# Autodesk Inventor assembly: ASY TZS FDS way1_940
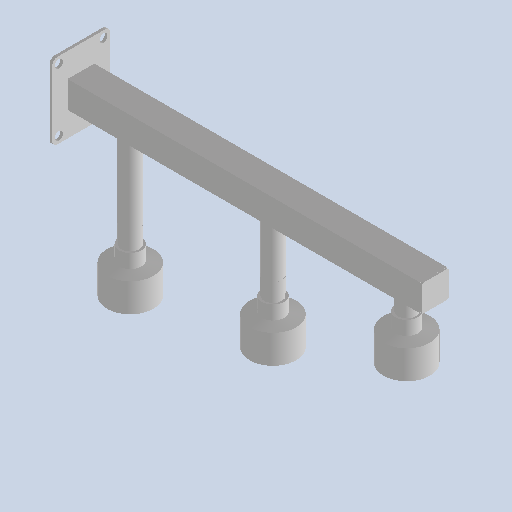
[picture p0: Inventor's stored thumbnail of the model, 512x512]
Saved by Autodesk Inventor 2025 (Build 290162010, 162A)
## iProperties
Created: 2025-07-02
Part Number: ASY TZS FDS way1_940
Document SubType Name: Assembly
Designer: admin
Author: user
## Documents named in this file (8)
- C:\Users\pokla\Documents\Inventor\TZS-Tazovskiy\Filter D940\FDS 940\ASY TZS FDS way1_940.iam
- C:\Users\pokla\Documents\Inventor\TZS-Tazovskiy\Filter D940\FDS 940\TZS 1661 FDS 940 way tube 1.ipt
- C:\Users\pokla\Documents\Inventor\TZS-Tazovskiy\Filter D940\FDS 940\TZS dummy filter element_940.ipt
- C:\Users\pokla\Documents\Inventor\TZS-Tazovskiy\Filter D940\FDS 940\TZS dummy pipe nippel_940.ipt
- C:\Users\pokla\Documents\Inventor\TZS-Tazovskiy\Filter D940\FDS 940\TZS 1684 FDS 940 way tube 4.ipt
- C:\Users\pokla\Documents\Inventor\TZS-Tazovskiy\Filter D940\FDS 940\TZS 1686 FDS 940 way tube 6.ipt
- C:\Users\pokla\Documents\Inventor\TZS-Tazovskiy\Filter D940\FDS 940\TZS 1669 FDS 940 FLANGE 3.ipt
- C:\Users\pokla\Documents\Inventor\TZS-Tazovskiy\Filter D940\FDS 940\TZS 1666 FDS 940 CUP 1.ipt
## Components (11 placed, 7 different names)
1. TZS 1661 FDS 940 way tube 1.ipt:1 — Rigid:2, Rigid:5, Rigid:10, Rigid:12, Rigid:13
2. TZS dummy filter element_940.ipt:1 — Rigid:1
3. TZS dummy pipe nippel_940.ipt:1 — Rigid:2, Rigid:1
4. TZS 1684 FDS 940 way tube 4.ipt:1 — Rigid:5, Rigid:4
5. TZS dummy filter element_940.ipt:2 — Rigid:3
6. TZS dummy pipe nippel_940.ipt:2 — Rigid:4, Rigid:3
7. TZS 1686 FDS 940 way tube 6.ipt:1 — Rigid:10, Rigid:7
8. TZS dummy filter element_940.ipt:3 — Rigid:6
9. TZS dummy pipe nippel_940.ipt:3 — Rigid:7, Rigid:6
10. TZS 1669 FDS 940 FLANGE 3.ipt:1 — Rigid:12
11. TZS 1666 FDS 940 CUP 1.ipt:1 — Rigid:13
## Relationships (10: WeldJoint 10)
- Rigid:2 [WeldJoint]: TZS 1661 FDS 940 way tube 1.ipt:1 ↔ TZS dummy pipe nippel_940.ipt:1
- Rigid:1 [WeldJoint]: TZS dummy filter element_940.ipt:1 ↔ TZS dummy pipe nippel_940.ipt:1
- Rigid:5 [WeldJoint]: TZS 1661 FDS 940 way tube 1.ipt:1 ↔ TZS 1684 FDS 940 way tube 4.ipt:1
- Rigid:4 [WeldJoint]: TZS 1684 FDS 940 way tube 4.ipt:1 ↔ TZS dummy pipe nippel_940.ipt:2
- Rigid:3 [WeldJoint]: TZS dummy filter element_940.ipt:2 ↔ TZS dummy pipe nippel_940.ipt:2
- Rigid:10 [WeldJoint]: TZS 1661 FDS 940 way tube 1.ipt:1 ↔ TZS 1686 FDS 940 way tube 6.ipt:1
- Rigid:7 [WeldJoint]: TZS 1686 FDS 940 way tube 6.ipt:1 ↔ TZS dummy pipe nippel_940.ipt:3
- Rigid:6 [WeldJoint]: TZS dummy filter element_940.ipt:3 ↔ TZS dummy pipe nippel_940.ipt:3
- Rigid:12 [WeldJoint] (-2 mm): TZS 1661 FDS 940 way tube 1.ipt:1 ↔ TZS 1669 FDS 940 FLANGE 3.ipt:1
- Rigid:13 [WeldJoint]: TZS 1661 FDS 940 way tube 1.ipt:1 ↔ TZS 1666 FDS 940 CUP 1.ipt:1
